# Autodesk Inventor assembly: GalvoandK1s4
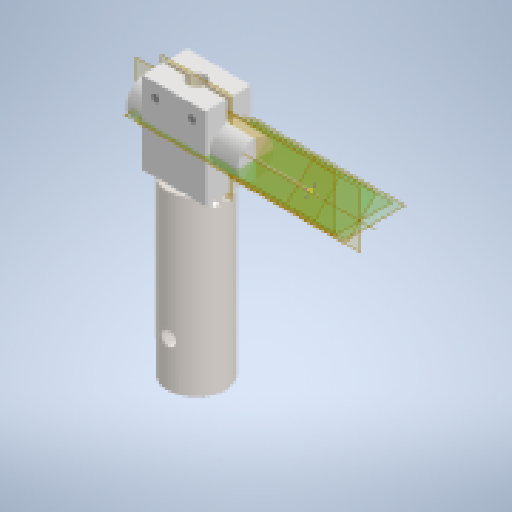
[picture p0: Inventor's stored thumbnail of the model, 512x512]
Saved by Autodesk Inventor 2025.2 (Build 292293000, 293)
## iProperties
Created: 2026-03-02
Part Number: GalvoandK1s4
Document SubType Name: Assembly
Designer: monolithic
Author: monolithic
## Documents named in this file (4)
- C:\Users\monolithic\Documents\GitHub\navigate-hardware\downloads\ASLM_CTASLM_Baseplate\CAD Assemblies\Powell ASLM\GalvoandK1s4.iam
- C:\Users\monolithic\Documents\GitHub\navigate-hardware\downloads\ASLM_CTASLM_Baseplate\CAD Assemblies\Powell ASLM\Galvo-Holder-PolarisMount_metal_v2.ipt
- C:\Users\monolithic\Documents\GitHub\navigate-hardware\downloads\ASLM_CTASLM_Baseplate\CAD Assemblies\Powell ASLM\Galvo_Galvo_Tilted.iam
- C:\Users\monolithic\Documents\GitHub\navigate-hardware\downloads\ASLM_CTASLM_Baseplate\CAD Assemblies\Powell ASLM\PLS-P3.ipt
## Components (3 placed, 3 different names)
1. Galvo-Holder-PolarisMount_metal_v2:1
2. Galvo_Galvo_Tilted:1 [sub-assembly]
3. PLS-P3:1
## Relationships (4: Mate 3, Angle 1)
- [Mate]: Galvo-Holder-PolarisMount_metal_v2:1 ↔ Galvo_Galvo_Tilted:1
- [Angle] (135 deg): Galvo-Holder-PolarisMount_metal_v2:1 ↔ Galvo_Galvo_Tilted:1
- [Mate]: Galvo-Holder-PolarisMount_metal_v2:1 ↔ PLS-P3:1
- [Mate]: Galvo-Holder-PolarisMount_metal_v2:1 ↔ PLS-P3:1
